# Autodesk Inventor assembly: Car_Assembly
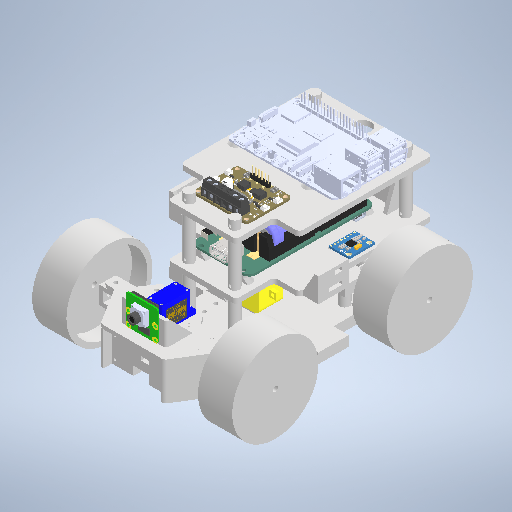
[picture p0: Inventor's stored thumbnail of the model, 512x512]
Saved by Autodesk Inventor 2025 (Build 290162010, 162A)
## iProperties
Created: 2024-05-24
Part Number: Car_Assembly
Document SubType Name: Assembly
Designer: Garfieldcmix
Author: Garfieldcmix
## Documents named in this file (35)
- C:\Users\DELL\Desktop\WRO-2024-CAD\Inventor\Car_Assembly.iam
- C:\Users\DELL\Desktop\WRO-2024-CAD\Inventor\SG90 - Micro Servo 9g - Tower Pro\SG90 - Micro Servo 9g - Tower Pro.iam
- C:\Users\DELL\Desktop\WRO-2024-CAD\Inventor\Front_Bridge.ipt
- C:\Users\DELL\Desktop\WRO-2024-CAD\Inventor\Front_Wheel_Anchor.ipt
- C:\Users\DELL\Desktop\WRO-2024-CAD\Inventor\Front_Wheel_Anchor_MIR.ipt
- C:\Users\DELL\Desktop\WRO-2024-CAD\Inventor\Wheel.ipt
- C:\Users\DELL\Desktop\WRO-2024-CAD\Inventor\Wheel_MIR.ipt
- C:\Users\DELL\Desktop\WRO-2024-CAD\Inventor\Pi camera module3\Pi camera module3.ipt
- C:\Users\DELL\Desktop\WRO-2024-CAD\Inventor\4519 DkStone Technic Axle 3\4519 DkStone Technic Axle 3.ipt
- C:\Users\DELL\Desktop\WRO-2024-CAD\Inventor\TT Motor\TT Motor.ipt
- C:\Users\DELL\Desktop\WRO-2024-CAD\Inventor\Lower_Chassis.ipt
- C:\Users\DELL\Desktop\WRO-2024-CAD\Inventor\Motor_Lego_Axle_Connector.ipt
- C:\Users\DELL\Desktop\WRO-2024-CAD\Inventor\Wheel_Lego_Axle_Connector.ipt
- C:\Users\DELL\Desktop\WRO-2024-CAD\Inventor\Front_Bridge_2.ipt
- C:\Users\DELL\Desktop\WRO-2024-CAD\Inventor\Servo_Steering_Linkage.ipt
- C:\Users\DELL\Desktop\WRO-2024-CAD\Inventor\hc-sr04\hc-sr04.iam
- C:\Users\DELL\Desktop\WRO-2024-CAD\Inventor\Lego_Frame_Holder.ipt
- C:\Users\DELL\Desktop\WRO-2024-CAD\Inventor\Lego_Frame_Holder_Extra.ipt
- C:\Users\DELL\Desktop\WRO-2024-CAD\Inventor\Lego_Frame_Holder_Extra_2.ipt
- C:\Users\DELL\Desktop\WRO-2024-CAD\Inventor\1.5_base.ipt
- C:\Users\DELL\Desktop\WRO-2024-CAD\Inventor\18650 2-WAY v5\18650 2-WAY v5.iam
- C:\Users\DELL\Desktop\WRO-2024-CAD\Inventor\MAKER-DRIVE\MAKER-DRIVE.iam
- C:\Users\DELL\Desktop\WRO-2024-CAD\Inventor\MPU_6050\MPU_6050.iam
- C:\Users\DELL\Desktop\WRO-2024-CAD\Inventor\RASPBERRY_PI_5\RASPBERRY_PI_5.iam
- C:\Users\DELL\Desktop\WRO-2024-CAD\Inventor\arduino nano\arduino nano.iam
- C:\Users\DELL\Desktop\WRO-2024-CAD\Inventor\Lego-Frame-Holder-Extra-Extra.ipt
- C:\Users\DELL\Desktop\WRO-2024-CAD\Inventor\SG90_Horn.ipt
- C:\Users\DELL\Desktop\WRO-2024-CAD\Inventor\2_Base.ipt
- C:\Users\DELL\Desktop\WRO-2024-CAD\Inventor\Wheel_Lego_Axle_Connector_2.ipt
- C:\Users\DELL\Desktop\WRO-2024-CAD\Inventor\diff_gear_holder.ipt
- C:\Users\DELL\Desktop\WRO-2024-CAD\Inventor\diff_gear_holder_3.ipt
- C:\Users\DELL\Desktop\WRO-2024-CAD\Inventor\diff_gear_holder_2.ipt
- C:\Users\DELL\Desktop\WRO-2024-CAD\Inventor\diff_gear_holder_4.ipt
- C:\Users\DELL\Desktop\WRO-2024-CAD\Inventor\Lower_Chassis_Pin_1.ipt
- C:\Users\DELL\Desktop\WRO-2024-CAD\Inventor\Lower_Chassis_Pin_2.ipt
## Components (52 placed, 39 different names)
1. Lower_Chassis_Pin_2:2 — Mate:268, Mate:269, Mate:113, Mate:115
2. Pi camera module3:1 — Mate:73, Mate:72, Mate:74
3. hc-sr04:1 [sub-assembly] — Mate:92, Mate:93, Mate:94
4. SG90_Servo [sub-assembly] — Mate:1, Mate:16, Mate:69, Mate:137, Mate:138
5. SG90_Horn:1 — Mate:137, Mate:138, Mate:139, Mate:141, Mate:201
6. Left_Servo_Steering_Linkage — Mate:85, Mate:83, Mate:139, Mate:141, Mate:202
7. Right_Servo_Steering_Linkage — Mate:199, Mate:200, Mate:201, Mate:202
8. Front_Bridge:1 — Mate:38, Mate:39, Mate:40, Mate:41, Mate:42, Mate:66, Mate:67, Mate:68, Mate:75, Mate:76, Mate:79, Mate:80, Angle:1, Mate:92, Mate:93, Mate:94
9. Front_Bridge_2:1 — Mate:66, Mate:67, Mate:68, Mate:69, Mate:73, Mate:72, Mate:74, Mate:1, Mate:16
10. Left_Front_Wheel_Anchor — Mate:75, Mate:76, Mate:77, Flush:84, Mate:85, Mate:83, Angle:1
11. Left_Front_Wheel — Mate:77, Flush:84
12. Right_Front_Wheel_Anchor — Mate:79, Mate:80, Mate:81, Flush:83, Mate:199, Mate:200
13. Right_Front_Wheel — Mate:81, Flush:83
14. Lower_Chassis:1 — Mate:38, Mate:39, Mate:40, Mate:41, Mate:42, Mate:57, Mate:91, Mate:119, Mate:120, Mate:122, Mate:123, Mate:229, Mate:230, Mate:231, Mate:232, Mate:233, Mate:234, Mate:245, Mate:246, Mate:247, Mate:253, Mate:255, Mate:256, Mate:257, Mate:258, Mate:259, Mate:262, Mate:263, Mate:264, Mate:265, Mate:266, Mate:267, Mate:268, Mate:269
15. TT Motor:1 — Mate:51, Mate:52, Mate:57, Mate:91, Mate:234
16. Motor_Lego_Axle_Connector — Mate:51, Mate:52, Mate:53, Mate:54
17. Lego_Driving_Shaft_Axle — Mate:53, Mate:54
18. diff_gear_holder:1 — Mate:229, Mate:230, Mate:231, Mate:232, Mate:233, Mate:235, Mate:236, Mate:237, Mate:238, Mate:239, Mate:240, Mate:248, Mate:249
19. diff_gear_holder_3:1 — Mate:235, Mate:236, Mate:237, Mate:241, Mate:242
20. diff_gear_holder_3:2 — Mate:238, Mate:239, Mate:240, Mate:243, Mate:244
21. diff_gear_holder_2:1 — Mate:241, Mate:242, Mate:250, Mate:252
22. diff_gear_holder_4:1 — Mate:245, Mate:246, Mate:247, Mate:248, Mate:249, Mate:250, Mate:251, Mate:253, Mate:254, Mate:255, Mate:256
23. Left_Wheel_Lego_Axle_Connector — Mate:219, Mate:220, Mate:221, Mate:251, Mate:252
24. Left_Wheel_Lego_Axle_Connector_2 — Mate:219, Mate:220, Mate:221, Mate:222, Mate:223
25. Left_Back_Wheel — Mate:222, Mate:223
26. diff_gear_holder_2:2 — Mate:243, Mate:244, Mate:261
27. diff_gear_holder_4:2 — Mate:257, Mate:258, Mate:259, Mate:260
28. Right_Wheel_Lego_Axle_Connector — Mate:224, Mate:225, Mate:226, Mate:260, Mate:261
29. Right_Wheel_Lego_Axle_Connector_2 — Mate:224, Mate:225, Mate:226, Mate:227, Mate:228
30. Right_Back_Wheel — Mate:227, Mate:228
31. Lower_Chassis_Pin_1:1 — Mate:262, Mate:263, Mate:121
32. Lower_Chassis_Pin_1:2 — Mate:264, Mate:265, Mate:124
33. Lower_Chassis_Pin_2:1 — Mate:266, Mate:267, Mate:254, Mate:116, Mate:118
34. Lego_Frame_Holder_Extra:1 — Mate:113, Mate:115, Mate:147, Mate:185, Mate:133, Mate:203
35. Lego_Frame_Holder_Extra:2 — Mate:116, Mate:118, Mate:125, Mate:128, Mate:187, Mate:188, Mate:204
36. Lego_Frame_Holder_Extra_2:1 — Mate:119, Mate:120, Mate:121, Mate:148, Mate:193, Mate:194, Mate:206
37. Lego_Frame_Holder_Extra_2:2 — Mate:122, Mate:123, Mate:124, Mate:126, Mate:149, Mate:191, Mate:192, Mate:205
38. 1.5_Base:1 — Mate:125, Mate:126, Mate:128, Mate:147, Mate:148, Mate:149, Mate:163, Mate:164, Mate:165, Mate:166, Mate:167, Mate:168, Mate:169, Mate:170, Mate:171, Mate:172, Mate:173
39. 18650 2-WAY v5:2 [sub-assembly] — Mate:164, Mate:165, Mate:166, Mate:167, Mate:173
40. MPU_6050:1 [sub-assembly] — Mate:163
41. arduino nano:1 [sub-assembly] — Mate:168, Mate:169, Mate:170, Mate:171, Mate:172
42. Lego-Frame-Holder-Extra-Extra:1 — Mate:185, Mate:133, Mate:146, Mate:186, Mate:203, Mate:216, Mate:218
43. Lego-Frame-Holder-Extra-Extra:2 — Mate:187, Mate:188, Mate:189, Mate:190, Mate:204, Mate:213, Mate:215
44. Lego-Frame-Holder-Extra-Extra:3 — Mate:191, Mate:192, Mate:195, Mate:196, Mate:205, Mate:210, Mate:212
45. Lego-Frame-Holder-Extra-Extra:4 — Mate:193, Mate:194, Mate:197, Mate:198, Mate:206, Mate:207, Mate:209
46. 2_Base:1 — Mate:146, Mate:151, Mate:152, Mate:153, Mate:154, Mate:155, Mate:156, Mate:157, Mate:158, Mate:159, Mate:160, Mate:186, Mate:189, Mate:190, Mate:195, Mate:196, Mate:197, Mate:198, Mate:208, Mate:211, Mate:214, Mate:217
47. RASPBERRY_PI_5:1 [sub-assembly] — Mate:151, Mate:152, Mate:153, Mate:154, Mate:155
48. MAKER-DRIVE:1 [sub-assembly] — Mate:156, Mate:157, Mate:158, Mate:159, Mate:160
49. Lego_Frame_Holder:7 — Mate:207, Mate:208, Mate:209
50. Lego_Frame_Holder:8 — Mate:210, Mate:211, Mate:212
51. Lego_Frame_Holder:9 — Mate:213, Mate:214, Mate:215
52. Lego_Frame_Holder:10 — Mate:216, Mate:217, Mate:218
## Relationships (162: Mate 159, Flush 2, Angle 1)
- Mate:1: SG90_Servo ↔ Front_Bridge_2:1
- Mate:16: SG90_Servo ↔ Front_Bridge_2:1
- Mate:38: Front_Bridge:1 ↔ Lower_Chassis:1
- Mate:39: Front_Bridge:1 ↔ Lower_Chassis:1
- Mate:40: Front_Bridge:1 ↔ Lower_Chassis:1
- Mate:41: Front_Bridge:1 ↔ Lower_Chassis:1
- Mate:42: Front_Bridge:1 ↔ Lower_Chassis:1
- Mate:51: TT Motor:1 ↔ Motor_Lego_Axle_Connector
- Mate:52: TT Motor:1 ↔ Motor_Lego_Axle_Connector
- Mate:53: Motor_Lego_Axle_Connector ↔ Lego_Driving_Shaft_Axle
- Mate:54: Motor_Lego_Axle_Connector ↔ Lego_Driving_Shaft_Axle
- Mate:57: Lower_Chassis:1 ↔ TT Motor:1
- Mate:66: Front_Bridge:1 ↔ Front_Bridge_2:1
- Mate:67: Front_Bridge:1 ↔ Front_Bridge_2:1
- Mate:68: Front_Bridge:1 ↔ Front_Bridge_2:1
- Mate:69: SG90_Servo ↔ Front_Bridge_2:1
- Mate:73: Pi camera module3:1 ↔ Front_Bridge_2:1
- Mate:72: Pi camera module3:1 ↔ Front_Bridge_2:1
- Mate:74: Pi camera module3:1 ↔ Front_Bridge_2:1
- Mate:75: Front_Bridge:1 ↔ Left_Front_Wheel_Anchor
- Mate:76: Front_Bridge:1 ↔ Left_Front_Wheel_Anchor
- Mate:77: Left_Front_Wheel_Anchor ↔ Left_Front_Wheel
- Flush:84: Left_Front_Wheel_Anchor ↔ Left_Front_Wheel
- Mate:79: Front_Bridge:1 ↔ Right_Front_Wheel_Anchor
- Mate:80: Front_Bridge:1 ↔ Right_Front_Wheel_Anchor
- Mate:81: Right_Front_Wheel_Anchor ↔ Right_Front_Wheel
- Flush:83: Right_Front_Wheel_Anchor ↔ Right_Front_Wheel
- Mate:85: Left_Servo_Steering_Linkage ↔ Left_Front_Wheel_Anchor
- Mate:83: Left_Servo_Steering_Linkage ↔ Left_Front_Wheel_Anchor
- Angle:1 (180 deg): Front_Bridge:1 ↔ Left_Front_Wheel_Anchor
- Mate:91: Lower_Chassis:1 ↔ TT Motor:1
- Mate:92: hc-sr04:1 ↔ Front_Bridge:1
- Mate:93: hc-sr04:1 ↔ Front_Bridge:1
- Mate:94: hc-sr04:1 ↔ Front_Bridge:1
- Mate:113: Lower_Chassis_Pin_2:2 ↔ Lego_Frame_Holder_Extra:1
- Mate:115: Lower_Chassis_Pin_2:2 ↔ Lego_Frame_Holder_Extra:1
- Mate:116: Lower_Chassis_Pin_2:1 ↔ Lego_Frame_Holder_Extra:2
- Mate:118: Lower_Chassis_Pin_2:1 ↔ Lego_Frame_Holder_Extra:2
- Mate:119: Lower_Chassis:1 ↔ Lego_Frame_Holder_Extra_2:1
- Mate:120: Lower_Chassis:1 ↔ Lego_Frame_Holder_Extra_2:1
- Mate:121: Lower_Chassis_Pin_1:1 ↔ Lego_Frame_Holder_Extra_2:1
- Mate:122: Lower_Chassis:1 ↔ Lego_Frame_Holder_Extra_2:2
- Mate:123: Lower_Chassis:1 ↔ Lego_Frame_Holder_Extra_2:2
- Mate:124: Lower_Chassis_Pin_1:2 ↔ Lego_Frame_Holder_Extra_2:2
- Mate:125: Lego_Frame_Holder_Extra:2 ↔ 1.5_Base:1
- Mate:126: Lego_Frame_Holder_Extra_2:2 ↔ 1.5_Base:1
- Mate:185: Lego_Frame_Holder_Extra:1 ↔ Lego-Frame-Holder-Extra-Extra:1
- Mate:133: Lego_Frame_Holder_Extra:1 ↔ Lego-Frame-Holder-Extra-Extra:1
- Mate:128: Lego_Frame_Holder_Extra:2 ↔ 1.5_Base:1
- Mate:137: SG90_Servo ↔ SG90_Horn:1
- Mate:138: SG90_Servo ↔ SG90_Horn:1
- Mate:139: SG90_Horn:1 ↔ Left_Servo_Steering_Linkage
- Mate:141: SG90_Horn:1 ↔ Left_Servo_Steering_Linkage
- Mate:146: Lego-Frame-Holder-Extra-Extra:1 ↔ 2_Base:1
- Mate:147: Lego_Frame_Holder_Extra:1 ↔ 1.5_Base:1
- Mate:148: Lego_Frame_Holder_Extra_2:1 ↔ 1.5_Base:1
- Mate:149: Lego_Frame_Holder_Extra_2:2 ↔ 1.5_Base:1
- Mate:151: 2_Base:1 ↔ RASPBERRY_PI_5:1
- Mate:152: 2_Base:1 ↔ RASPBERRY_PI_5:1
- Mate:153: 2_Base:1 ↔ RASPBERRY_PI_5:1
- Mate:154: 2_Base:1 ↔ RASPBERRY_PI_5:1
- Mate:155: 2_Base:1 ↔ RASPBERRY_PI_5:1
- Mate:156: 2_Base:1 ↔ MAKER-DRIVE:1
- Mate:157: 2_Base:1 ↔ MAKER-DRIVE:1
- Mate:158: 2_Base:1 ↔ MAKER-DRIVE:1
- Mate:159: 2_Base:1 ↔ MAKER-DRIVE:1
- Mate:160: 2_Base:1 ↔ MAKER-DRIVE:1
- Mate:163: 1.5_Base:1 ↔ MPU_6050:1
- Mate:164: 1.5_Base:1 ↔ 18650 2-WAY v5:2
- Mate:165: 1.5_Base:1 ↔ 18650 2-WAY v5:2
- Mate:166: 1.5_Base:1 ↔ 18650 2-WAY v5:2
- Mate:167: 1.5_Base:1 ↔ 18650 2-WAY v5:2
- Mate:168: 1.5_Base:1 ↔ arduino nano:1
- Mate:169: 1.5_Base:1 ↔ arduino nano:1
- Mate:170: 1.5_Base:1 ↔ arduino nano:1
- Mate:171: 1.5_Base:1 ↔ arduino nano:1
- Mate:172: 1.5_Base:1 ↔ arduino nano:1
- Mate:173: 1.5_Base:1 ↔ 18650 2-WAY v5:2
- Mate:186: Lego-Frame-Holder-Extra-Extra:1 ↔ 2_Base:1
- Mate:187: Lego_Frame_Holder_Extra:2 ↔ Lego-Frame-Holder-Extra-Extra:2
- Mate:188: Lego_Frame_Holder_Extra:2 ↔ Lego-Frame-Holder-Extra-Extra:2
- Mate:189: Lego-Frame-Holder-Extra-Extra:2 ↔ 2_Base:1
- Mate:190: Lego-Frame-Holder-Extra-Extra:2 ↔ 2_Base:1
- Mate:191: Lego_Frame_Holder_Extra_2:2 ↔ Lego-Frame-Holder-Extra-Extra:3
- Mate:192: Lego_Frame_Holder_Extra_2:2 ↔ Lego-Frame-Holder-Extra-Extra:3
- Mate:193: Lego_Frame_Holder_Extra_2:1 ↔ Lego-Frame-Holder-Extra-Extra:4
- Mate:194: Lego_Frame_Holder_Extra_2:1 ↔ Lego-Frame-Holder-Extra-Extra:4
- Mate:195: Lego-Frame-Holder-Extra-Extra:3 ↔ 2_Base:1
- Mate:196: Lego-Frame-Holder-Extra-Extra:3 ↔ 2_Base:1
- Mate:197: Lego-Frame-Holder-Extra-Extra:4 ↔ 2_Base:1
- Mate:198: Lego-Frame-Holder-Extra-Extra:4 ↔ 2_Base:1
- Mate:199: Right_Servo_Steering_Linkage ↔ Right_Front_Wheel_Anchor
- Mate:200: Right_Servo_Steering_Linkage ↔ Right_Front_Wheel_Anchor
- Mate:201: SG90_Horn:1 ↔ Right_Servo_Steering_Linkage
- Mate:202: Left_Servo_Steering_Linkage ↔ Right_Servo_Steering_Linkage
- Mate:203: Lego_Frame_Holder_Extra:1 ↔ Lego-Frame-Holder-Extra-Extra:1
- Mate:204: Lego_Frame_Holder_Extra:2 ↔ Lego-Frame-Holder-Extra-Extra:2
- Mate:205: Lego_Frame_Holder_Extra_2:2 ↔ Lego-Frame-Holder-Extra-Extra:3
- Mate:206: Lego_Frame_Holder_Extra_2:1 ↔ Lego-Frame-Holder-Extra-Extra:4
- Mate:207: Lego-Frame-Holder-Extra-Extra:4 ↔ Lego_Frame_Holder:7
- Mate:208: 2_Base:1 ↔ Lego_Frame_Holder:7
- Mate:209: Lego-Frame-Holder-Extra-Extra:4 ↔ Lego_Frame_Holder:7
- Mate:210: Lego-Frame-Holder-Extra-Extra:3 ↔ Lego_Frame_Holder:8
- Mate:211: 2_Base:1 ↔ Lego_Frame_Holder:8
- Mate:212: Lego-Frame-Holder-Extra-Extra:3 ↔ Lego_Frame_Holder:8
- Mate:213: Lego-Frame-Holder-Extra-Extra:2 ↔ Lego_Frame_Holder:9
- Mate:214: 2_Base:1 ↔ Lego_Frame_Holder:9
- Mate:215: Lego-Frame-Holder-Extra-Extra:2 ↔ Lego_Frame_Holder:9
- Mate:216: Lego-Frame-Holder-Extra-Extra:1 ↔ Lego_Frame_Holder:10
- Mate:217: 2_Base:1 ↔ Lego_Frame_Holder:10
- Mate:218: Lego-Frame-Holder-Extra-Extra:1 ↔ Lego_Frame_Holder:10
- Mate:219: Left_Wheel_Lego_Axle_Connector ↔ Left_Wheel_Lego_Axle_Connector_2
- Mate:220: Left_Wheel_Lego_Axle_Connector ↔ Left_Wheel_Lego_Axle_Connector_2
- Mate:221: Left_Wheel_Lego_Axle_Connector ↔ Left_Wheel_Lego_Axle_Connector_2
- Mate:222: Left_Wheel_Lego_Axle_Connector_2 ↔ Left_Back_Wheel
- Mate:223: Left_Wheel_Lego_Axle_Connector_2 ↔ Left_Back_Wheel
- Mate:224: Right_Wheel_Lego_Axle_Connector ↔ Right_Wheel_Lego_Axle_Connector_2
- Mate:225: Right_Wheel_Lego_Axle_Connector ↔ Right_Wheel_Lego_Axle_Connector_2
- Mate:226: Right_Wheel_Lego_Axle_Connector ↔ Right_Wheel_Lego_Axle_Connector_2
- Mate:227: Right_Wheel_Lego_Axle_Connector_2 ↔ Right_Back_Wheel
- Mate:228: Right_Wheel_Lego_Axle_Connector_2 ↔ Right_Back_Wheel
- Mate:229: Lower_Chassis:1 ↔ diff_gear_holder:1
- Mate:230: Lower_Chassis:1 ↔ diff_gear_holder:1
- Mate:231: Lower_Chassis:1 ↔ diff_gear_holder:1
- Mate:232: Lower_Chassis:1 ↔ diff_gear_holder:1
- Mate:233: Lower_Chassis:1 ↔ diff_gear_holder:1
- Mate:234: Lower_Chassis:1 ↔ TT Motor:1
- Mate:235: diff_gear_holder:1 ↔ diff_gear_holder_3:1
- Mate:236: diff_gear_holder:1 ↔ diff_gear_holder_3:1
- Mate:237: diff_gear_holder:1 ↔ diff_gear_holder_3:1
- Mate:238: diff_gear_holder:1 ↔ diff_gear_holder_3:2
- Mate:239: diff_gear_holder:1 ↔ diff_gear_holder_3:2
- Mate:240: diff_gear_holder:1 ↔ diff_gear_holder_3:2
- Mate:241: diff_gear_holder_3:1 ↔ diff_gear_holder_2:1
- Mate:242: diff_gear_holder_3:1 ↔ diff_gear_holder_2:1
- Mate:243: diff_gear_holder_3:2 ↔ diff_gear_holder_2:2
- Mate:244: diff_gear_holder_3:2 ↔ diff_gear_holder_2:2
- Mate:245: Lower_Chassis:1 ↔ diff_gear_holder_4:1
- Mate:246: Lower_Chassis:1 ↔ diff_gear_holder_4:1
- Mate:247: Lower_Chassis:1 ↔ diff_gear_holder_4:1
- Mate:248: diff_gear_holder:1 ↔ diff_gear_holder_4:1
- Mate:249: diff_gear_holder:1 ↔ diff_gear_holder_4:1
- Mate:250: diff_gear_holder_2:1 ↔ diff_gear_holder_4:1
- Mate:251: diff_gear_holder_4:1 ↔ Left_Wheel_Lego_Axle_Connector
- Mate:252: diff_gear_holder_2:1 ↔ Left_Wheel_Lego_Axle_Connector
- Mate:253: Lower_Chassis:1 ↔ diff_gear_holder_4:1
- Mate:254: diff_gear_holder_4:1 ↔ Lower_Chassis_Pin_2:1
- Mate:255: Lower_Chassis:1 ↔ diff_gear_holder_4:1
- Mate:256: Lower_Chassis:1 ↔ diff_gear_holder_4:1
- Mate:257: Lower_Chassis:1 ↔ diff_gear_holder_4:2
- Mate:258: Lower_Chassis:1 ↔ diff_gear_holder_4:2
- Mate:259: Lower_Chassis:1 ↔ diff_gear_holder_4:2
- Mate:260: diff_gear_holder_4:2 ↔ Right_Wheel_Lego_Axle_Connector
- Mate:261: diff_gear_holder_2:2 ↔ Right_Wheel_Lego_Axle_Connector
- Mate:262: Lower_Chassis:1 ↔ Lower_Chassis_Pin_1:1
- Mate:263: Lower_Chassis:1 ↔ Lower_Chassis_Pin_1:1
- Mate:264: Lower_Chassis:1 ↔ Lower_Chassis_Pin_1:2
- Mate:265: Lower_Chassis:1 ↔ Lower_Chassis_Pin_1:2
- Mate:266: Lower_Chassis:1 ↔ Lower_Chassis_Pin_2:1
- Mate:267: Lower_Chassis:1 ↔ Lower_Chassis_Pin_2:1
- Mate:268: Lower_Chassis_Pin_2:2 ↔ Lower_Chassis:1
- Mate:269: Lower_Chassis_Pin_2:2 ↔ Lower_Chassis:1
